# Autodesk Inventor assembly: arm standoff
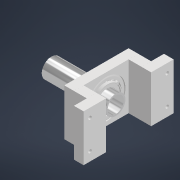
[picture p0: Inventor's stored thumbnail of the model, 180x180]
Saved by Autodesk Inventor 2022 (Build 260153000, 153)
## iProperties
Created: 2021-11-03
Part Number: arm standoff
Document SubType Name: Assembly
Designer: 17185
Author: 17185
## Documents named in this file (6)
- G:\__projects\ROBOTICS\RCR\v3\Chassis\arm standoff\arm standoff.iam
- G:\__projects\ROBOTICS\RCR\v3\Chassis\arm standoff\Part1.ipt
- G:\__projects\ROBOTICS\RCR\v3\Chassis\arm standoff\Part2.ipt
- G:\__projects\ROBOTICS\RCR\v3\Chassis\arm standoff\Part3.ipt
- G:\__projects\ROBOTICS\RCR\v3\Chassis\arm standoff\TubingForWires.ipt
- G:\__projects\ROBOTICS\RCR\v3\Chassis\arm standoff\5709K88_Tapered-Roller Bearing with Steel Ring.ipt
## Components (7 placed, 5 different names)
1. Part1:1 — Flush:2, Mate:1, Flush:3, Flush:4, Mate:2, Mate:5, Mate:7, Cylindrical:2, Mate:8
2. Part2:1 — Flush:2, Mate:1, Mate:3, Flush:5, Flush:6, Flush:9, Mate:5
3. Part2:2 — Flush:3, Flush:4, Mate:2, Flush:7, Mate:4, Flush:8
4. Part3:1 — Mate:3, Flush:5, Flush:6, Flush:9
5. Part3:2 — Flush:7, Mate:4, Flush:8, Flush:11
6. TubingForWires:1 — Flush:11, Mate:7, Cylindrical:1
7. 5709K88_Tapered-Roller Bearing with Steel Ring:1 — Cylindrical:1, Cylindrical:2, Mate:8
## Relationships (18: Flush 9, Mate 7, CylindricalJoint 2)
- Flush:2: Part1:1 ↔ Part2:1
- Mate:1: Part1:1 ↔ Part2:1
- Flush:3: Part1:1 ↔ Part2:2
- Flush:4: Part1:1 ↔ Part2:2
- Mate:2: Part1:1 ↔ Part2:2
- Mate:3: Part2:1 ↔ Part3:1
- Flush:5: Part2:1 ↔ Part3:1
- Flush:6: Part2:1 ↔ Part3:1
- Flush:7: Part2:2 ↔ Part3:2
- Mate:4: Part2:2 ↔ Part3:2
- Flush:8: Part2:2 ↔ Part3:2
- Flush:9: Part2:1 ↔ Part3:1
- Mate:5: Part1:1 ↔ Part2:1
- Flush:11 (25.4 mm): Part3:2 ↔ TubingForWires:1
- Mate:7: Part1:1 ↔ TubingForWires:1
- Cylindrical:1: TubingForWires:1 ↔ 5709K88_Tapered-Roller Bearing with Steel Ring:1
- Cylindrical:2: Part1:1 ↔ 5709K88_Tapered-Roller Bearing with Steel Ring:1
- Mate:8: Part1:1 ↔ 5709K88_Tapered-Roller Bearing with Steel Ring:1
